# Autodesk Inventor assembly: PZT Assembly Through
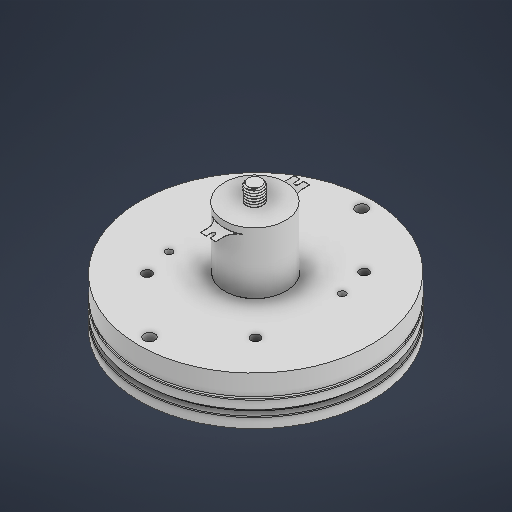
[picture p0: Inventor's stored thumbnail of the model, 512x512]
Saved by Autodesk Inventor 2025 (Build 290162000, 162)
## iProperties
Created: 2024-07-01
Part Number: PZT Assembly Through
Document SubType Name: Assembly
Designer: mayhe
Author: mayhe
## Documents named in this file (9)
- C:\Users\mayhe\OneDrive\Documents\GitHub\In-situ-monitoring-of-powder-bed-fusion-additive-manufacturing\system_development\Orichalcum\v0.2\Hardware_design\pzt-parts\PZT Assembly Through.iam
- C:\Users\mayhe\OneDrive\Documents\GitHub\In-situ-monitoring-of-powder-bed-fusion-additive-manufacturing\system_development\Orichalcum\v0.2\Hardware_design\pzt-parts\Modified Substrate Plate Bottom.ipt
- C:\Users\mayhe\OneDrive\Documents\GitHub\In-situ-monitoring-of-powder-bed-fusion-additive-manufacturing\system_development\Orichalcum\v0.2\Hardware_design\pzt-parts\shaker cut.ipt
- C:\Users\mayhe\OneDrive\Documents\GitHub\In-situ-monitoring-of-powder-bed-fusion-additive-manufacturing\system_development\Orichalcum\v0.2\Hardware_design\pzt-parts\Build Plateform.ipt
- C:\Users\mayhe\OneDrive\Documents\GitHub\In-situ-monitoring-of-powder-bed-fusion-additive-manufacturing\system_development\Orichalcum\v0.2\Hardware_design\pzt-parts\Clamp Ring.ipt
- C:\Users\mayhe\OneDrive\Documents\GitHub\In-situ-monitoring-of-powder-bed-fusion-additive-manufacturing\system_development\Orichalcum\v0.2\Hardware_design\pzt-parts\91294A208_Black-Oxide Alloy Steel Hex Drive F.ipt
- C:\Users\mayhe\OneDrive\Documents\GitHub\In-situ-monitoring-of-powder-bed-fusion-additive-manufacturing\system_development\Orichalcum\v0.2\Hardware_design\pzt-parts\91290.ipt
- C:\Users\mayhe\OneDrive\Documents\GitHub\In-situ-monitoring-of-powder-bed-fusion-additive-manufacturing\system_development\Orichalcum\v0.2\Hardware_design\pzt-parts\substrate plate 12mm hole.ipt
- C:\Users\mayhe\OneDrive\Documents\GitHub\In-situ-monitoring-of-powder-bed-fusion-additive-manufacturing\system_development\Orichalcum\v0.2\Hardware_design\pzt-parts\m12 91290.ipt
## Components (16 placed, 8 different names)
1. shaker cut:1 — Rotational:19, Mate:2
2. Build Plateform:1 — Mate:1, Rotational:3, Rotational:8
3. Clamp Ring:1 — Mate:1, Rotational:3, Rotational:9, Rotational:10, Rotational:11, Rotational:12, Rotational:13, Rotational:14, Rotational:15, Rotational:16
4. Modified Substrate Plate Bottom:3 — Rotational:8, Rotational:17, Rotational:18, Rotational:19, Rotational:20
5. substrate plate 12mm hole:1 — Mate:2
6. m12 91290:1 — Rotational:20
7. 91294A208_Black-Oxide Alloy Steel Hex Drive F:1 — Rotational:9
8. 91294A208_Black-Oxide Alloy Steel Hex Drive F:2 — Rotational:10
9. 91294A208_Black-Oxide Alloy Steel Hex Drive F:3 — Rotational:11
10. 91294A208_Black-Oxide Alloy Steel Hex Drive F:4 — Rotational:12
11. 91294A208_Black-Oxide Alloy Steel Hex Drive F:5 — Rotational:15
12. 91294A208_Black-Oxide Alloy Steel Hex Drive F:6 — Rotational:16
13. 91294A208_Black-Oxide Alloy Steel Hex Drive F:7 — Rotational:13
14. 91294A208_Black-Oxide Alloy Steel Hex Drive F:8 — Rotational:14
15. 91290:1 — Rotational:17
16. 91290:2 — Rotational:18
## Relationships (16: RevoluteJoint 14, Mate 2)
- Mate:1: Build Plateform:1 ↔ Clamp Ring:1
- Rotational:3 [RevoluteJoint]: Build Plateform:1 ↔ Clamp Ring:1
- Rotational:8 [RevoluteJoint]: Build Plateform:1 ↔ Modified Substrate Plate Bottom:3
- Rotational:9 [RevoluteJoint]: Clamp Ring:1 ↔ 91294A208_Black-Oxide Alloy Steel Hex Drive F:1
- Rotational:10 [RevoluteJoint]: Clamp Ring:1 ↔ 91294A208_Black-Oxide Alloy Steel Hex Drive F:2
- Rotational:11 [RevoluteJoint]: Clamp Ring:1 ↔ 91294A208_Black-Oxide Alloy Steel Hex Drive F:3
- Rotational:12 [RevoluteJoint]: Clamp Ring:1 ↔ 91294A208_Black-Oxide Alloy Steel Hex Drive F:4
- Rotational:13 [RevoluteJoint]: Clamp Ring:1 ↔ 91294A208_Black-Oxide Alloy Steel Hex Drive F:7
- Rotational:14 [RevoluteJoint]: Clamp Ring:1 ↔ 91294A208_Black-Oxide Alloy Steel Hex Drive F:8
- Rotational:15 [RevoluteJoint]: Clamp Ring:1 ↔ 91294A208_Black-Oxide Alloy Steel Hex Drive F:5
- Rotational:16 [RevoluteJoint]: Clamp Ring:1 ↔ 91294A208_Black-Oxide Alloy Steel Hex Drive F:6
- Rotational:17 [RevoluteJoint]: Modified Substrate Plate Bottom:3 ↔ 91290:1
- Rotational:18 [RevoluteJoint]: Modified Substrate Plate Bottom:3 ↔ 91290:2
- Rotational:19 [RevoluteJoint]: shaker cut:1 ↔ Modified Substrate Plate Bottom:3
- Mate:2: shaker cut:1 ↔ substrate plate 12mm hole:1
- Rotational:20 [RevoluteJoint]: Modified Substrate Plate Bottom:3 ↔ m12 91290:1
